# Autodesk Inventor assembly: Assembly_Final
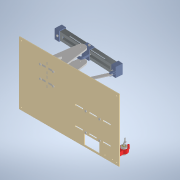
[picture p0: Inventor's stored thumbnail of the model, 180x180]
Saved by Autodesk Inventor 2022 (Build 260153000, 153)
## iProperties
Created: 2022-02-22
Part Number: Assembly_Final
Document SubType Name: Assembly
Designer: katha
Author: katha
## Documents named in this file (10)
- C:\Users\katha\OneDrive\Escritorio\Mini_Proyecto_Diseno\Diseno_18012\Modelo_MPD\Assembly_Final.iam
- C:\Users\katha\OneDrive\Escritorio\Mini_Proyecto_Diseno\Diseno_18012\Modelo_MPD\Acople_TransPot.ipt
- C:\Users\katha\OneDrive\Escritorio\Mini_Proyecto_Diseno\Diseno_18012\Modelo_MPD\Eslabon_TransPot.ipt
- C:\Users\katha\OneDrive\Escritorio\Mini_Proyecto_Diseno\Diseno_18012\Modelo_MPD\Base_proyecto.ipt
- C:\Users\katha\OneDrive\Escritorio\Mini_Proyecto_Diseno\Diseno_18012\Modelo_MPD\Base_Soporte.ipt
- C:\Users\katha\OneDrive\Escritorio\Mini_Proyecto_Diseno\Diseno_18012\Modelo_MPD\Base.ipt
- C:\Users\katha\OneDrive\Escritorio\Mini_Proyecto_Diseno\Diseno_18012\Modelo_MPD\Carril.iam
- C:\Users\katha\OneDrive\Escritorio\Mini_Proyecto_Diseno\Diseno_18012\Modelo_MPD\M4_short.ipt
- C:\Users\katha\OneDrive\Escritorio\Mini_Proyecto_Diseno\Diseno_18012\Modelo_MPD\motor.ipt
- C:\Users\katha\OneDrive\Escritorio\Mini_Proyecto_Diseno\Diseno_18012\Modelo_MPD\base_motor.ipt
## Components (18 placed, 9 different names)
1. Base_proyecto:1 — Flush:1, Mate:10, Flush:13, Mate:26, Mate:27, Mate:28, Mate:29, Mate:30, Mate:31, Mate:32, Mate:33, Mate:34, Mate:35, Mate:36, Mate:37, Mate:38, Mate:39, Mate:40, Mate:41, Flush:16
2. Base_Soporte:2 — Mate:6, Mate:7, Flush:4, Mate:8, Mate:9, Flush:5, Flush:13
3. Base:1 — Mate:6, Mate:7, Flush:4, Mate:10, Mate:14
4. Base:2 — Mate:8, Mate:9, Flush:5, Mate:11
5. Carril:1 [sub-assembly] — Mate:11, Mate:14, Mate:20, Mate:21
6. Acople_TransPot:1 — Mate:18, Mate:19
7. Eslabon_TransPot:1 — Mate:18, Mate:19, Mate:20, Mate:21
8. M4_short:1 — Mate:26, Mate:27
9. M4_short:2 — Mate:28, Mate:35
10. M4_short:3 — Mate:29, Mate:36
11. M4_short:4 — Mate:30, Mate:37
12. M4_short:5 — Mate:31, Mate:41
13. M4_short:6 — Mate:33, Mate:39
14. M4_short:7 — Mate:32, Mate:38
15. M4_short:8 — Mate:34, Mate:40
16. M4_short:9
17. motor:1 — Mate:45, Flush:15
18. base_motor:1 — Mate:45, Flush:15, Flush:16
## Relationships (34: Mate 28, Flush 6)
- Flush:1: Base_proyecto:1
- Mate:6: Base_Soporte:2 ↔ Base:1
- Mate:7: Base_Soporte:2 ↔ Base:1
- Flush:4: Base_Soporte:2 ↔ Base:1
- Mate:8: Base_Soporte:2 ↔ Base:2
- Mate:9: Base_Soporte:2 ↔ Base:2
- Flush:5: Base_Soporte:2 ↔ Base:2
- Mate:10: Base_proyecto:1 ↔ Base:1
- Mate:11: Base:2 ↔ Carril:1
- Mate:14 (18.25 mm): Base:1 ↔ Carril:1
- Mate:18: Acople_TransPot:1 ↔ Eslabon_TransPot:1
- Mate:19: Acople_TransPot:1 ↔ Eslabon_TransPot:1
- Mate:20 (0.3 mm): Carril:1 ↔ Eslabon_TransPot:1
- Mate:21: Carril:1 ↔ Eslabon_TransPot:1
- Flush:13 (110 mm): Base_proyecto:1 ↔ Base_Soporte:2
- Mate:26: Base_proyecto:1 ↔ M4_short:1
- Mate:27: Base_proyecto:1 ↔ M4_short:1
- Mate:28: Base_proyecto:1 ↔ M4_short:2
- Mate:29: Base_proyecto:1 ↔ M4_short:3
- Mate:30: Base_proyecto:1 ↔ M4_short:4
- Mate:31: Base_proyecto:1 ↔ M4_short:5
- Mate:32: Base_proyecto:1 ↔ M4_short:7
- Mate:33: Base_proyecto:1 ↔ M4_short:6
- Mate:34: Base_proyecto:1 ↔ M4_short:8
- Mate:35: Base_proyecto:1 ↔ M4_short:2
- Mate:36: Base_proyecto:1 ↔ M4_short:3
- Mate:37: Base_proyecto:1 ↔ M4_short:4
- Mate:38: Base_proyecto:1 ↔ M4_short:7
- Mate:39: Base_proyecto:1 ↔ M4_short:6
- Mate:40: Base_proyecto:1 ↔ M4_short:8
- Mate:41: Base_proyecto:1 ↔ M4_short:5
- Mate:45: motor:1 ↔ base_motor:1
- Flush:15 (-4 mm): motor:1 ↔ base_motor:1
- Flush:16: Base_proyecto:1 ↔ base_motor:1
